# Autodesk Inventor assembly: 000 Ensamblaje hw_DAA - panel - BASIC
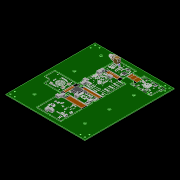
[picture p0: Inventor's stored thumbnail of the model, 180x180]
Saved by Autodesk Inventor 2018 (Build 220112000, 112)
## iProperties
Created: 2024-08-29
Part Number: 000 Ensamblaje hw_DAA - panel - BASIC
Document SubType Name: Assembly
Designer: cda1
Author: cda1
## Documents named in this file (3)
- C:\Users\cda1\Git\DAA\items\hw_DAA\items\3d_DAA_panel\variants\BASIC\3d\000 Ensamblaje hw_DAA - panel - BASIC.iam
- C:\Users\cda1\Git\DAA\items\hw_DAA\variants\BASIC\3d\En plano\Dummy\hw_DAA - BASIC - plano - dummy.ipt
- C:\Users\cda1\Git\DAA\items\hw_DAA\items\3d_DAA_panel\3d\3d_DAA_panel - Panel.ipt
## Components (2 placed, 2 different names)
1. hw_DAA - BASIC - plano - dummy:1 — Nivelación:1, Coincidencia:1, Coincidencia:2
2. 3d_DAA_panel - Panel:1 — Nivelación:1, Coincidencia:1, Coincidencia:2
## Relationships (3: Mate 2, Flush 1)
- Nivelación:1 [Flush]: hw_DAA - BASIC - plano - dummy:1 ↔ 3d_DAA_panel - Panel:1
- Coincidencia:1 [Mate]: hw_DAA - BASIC - plano - dummy:1 ↔ 3d_DAA_panel - Panel:1
- Coincidencia:2 [Mate]: hw_DAA - BASIC - plano - dummy:1 ↔ 3d_DAA_panel - Panel:1
